# Autodesk Inventor assembly: EvelFrontFrame
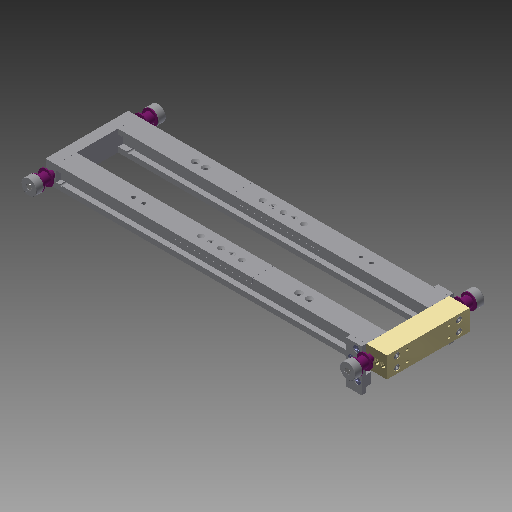
[picture p0: Inventor's stored thumbnail of the model, 512x512]
Saved by Autodesk Inventor 2019 (Build 230136000, 136)
## iProperties
Created: 2019-09-29
Part Number: EvelFrontFrame
Document SubType Name: Weldment
Designer: james
Weld Material: Welded Aluminum-6061
Author: james
## Documents named in this file (4)
- F:\JimsDesign\Jims2020FTC\EvelFrontFrame.iam
- F:\JimsDesign\Jims2020FTC\ElevatorFrame.iam
- F:\JimsDesign\Jims2020FTC\SliderRight.iam
- F:\JimsDesign\Jims2020FTC\FullElevatorShart.iam
## Components (5 placed, 3 different names)
1. ElevatorFrame:1 [sub-assembly] — Mate:1, Mate:11, Mate:12, Mate:13, Mate:14, Mate:15, Mate:16, Mate:17, Mate:18, Mate:19
2. SliderRight:1 [sub-assembly] — Mate:13, Mate:14, Mate:15
3. FullElevatorShart:1 [sub-assembly] — Mate:12, Mate:19
4. FullElevatorShart:2 [sub-assembly] — Mate:1, Mate:11
5. SliderRight:2 [sub-assembly] — Mate:16, Mate:17, Mate:18
## Relationships (10: Mate 10)
- Mate:1: ElevatorFrame:1 ↔ FullElevatorShart:2
- Mate:11: ElevatorFrame:1 ↔ FullElevatorShart:2
- Mate:12: ElevatorFrame:1 ↔ FullElevatorShart:1
- Mate:13: ElevatorFrame:1 ↔ SliderRight:1
- Mate:14: ElevatorFrame:1 ↔ SliderRight:1
- Mate:15: ElevatorFrame:1 ↔ SliderRight:1
- Mate:16: ElevatorFrame:1 ↔ SliderRight:2
- Mate:17: ElevatorFrame:1 ↔ SliderRight:2
- Mate:18: ElevatorFrame:1 ↔ SliderRight:2
- Mate:19: ElevatorFrame:1 ↔ FullElevatorShart:1
